# Autodesk Inventor assembly: ствол и крышка
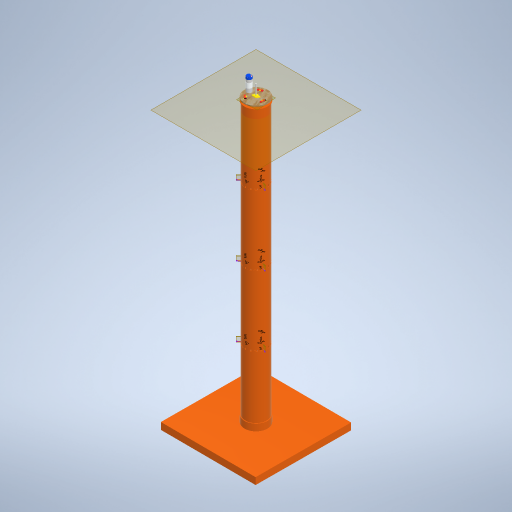
[picture p0: Inventor's stored thumbnail of the model, 512x512]
Saved by Autodesk Inventor 2023 (Build 270158000, 158)
## iProperties
Created: 2023-12-24
Part Number: ствол и крышка
Document SubType Name: Assembly
Designer: Dell
Author: Dell
## Documents named in this file (17)
- C:\Fox_Crow\Work\Crow_Sborka\ствол и крышка.iam
- C:\Fox_Crow\Work\Crow_Sborka\Поворотный механизм\Pitsco Education-739085.ipt
- C:\Fox_Crow\Work\Crow_Sborka\Поворотный механизм\Cap_pipes.ipt
- C:\Fox_Crow\Work\Crow_Sborka\Поворотный механизм\Pitsco Education-739028.ipt
- C:\Fox_Crow\Work\Crow_Sborka\Поворотный механизм\Fanerka.ipt
- C:\Fox_Crow\Work\Crow_Sborka\Поворотный механизм\Prostavka.ipt
- C:\Fox_Crow\Work\Crow_Sborka\Поворотный механизм\Det_podsh.ipt
- C:\Fox_Crow\Work\Crow_Sborka\Поворотный механизм\Podsh.ipt
- C:\Fox_Crow\Work\Crow_Sborka\Поворотный механизм\User Library-Bearing KFL08.ipt
- C:\Fox_Crow\Work\Crow_Sborka\Поворотный механизм\trubka.ipt
- C:\Users\Dell\Downloads\User Library-DC gearhead motor.ipt
- C:\Fox_Crow\Work\Crow_Sborka\Поворотный механизм\39079_TXM-Motor Shaft Hub With Set Screw.ipt
- C:\Fox_Crow\Work\Crow_Sborka\Поворотный механизм\SHF8 Горизонтальный держатель вала.ipt
- C:\Fox_Crow\Work\Crow_Sborka\Поворотный механизм\ISO 14583 — M5x16-4.8.ipt
- C:\Fox_Crow\Work\Crow_Sborka\Поворотный механизм\ISO 7046-1 - M6 x 20_ - 4.8 - H - ISO.ipt
- C:\Fox_Crow\Work\Crow_Sborka\Поворотный механизм\44260_txm torquenado dc motor.ipt
- C:\Fox_Crow\Work\Crow_Sborka\Ствол.iam
## Components (24 placed, 16 different names)
1. Pitsco Education-739085:1 — Жесткий:6, Совмещение:10, Совмещение:11, Совмещение:13, Совмещение:16
2. Cap_pipes:1 — Цилиндрический:2, Совмещение:8, Совмещение:9, Жесткий:9
3. Pitsco Education-739028:1
4. Fanerka:1 — Совмещение:9, Плоский:1, Плоский:2, Плоский:3, Цилиндрический:4, С поворотом:3, С поворотом:4, Жесткий:8
5. Prostavka:1 — Цилиндрический:2, Совмещение:8, Жесткий:5
6. User Library-Bearing KFL08:1 — С поворотом:3, С поворотом:4
7. trubka:1 — Жесткий:5, Жесткий:6, Цилиндрический:5
8. User Library-DC gearhead motor:1 — Цилиндрический:4, Жесткий:7
9. 39079_TXM-Motor Shaft Hub With Set Screw:1 — Жесткий:7
10. Винт ISO 14583:2011(E) M5x16-4.8:2
11. Винт ISO 14583:2011(E) M5x16-4.8:3
12. SHF8 Горизонтальный держатель вала:3 — Цилиндрический:5
13. ISO 7046-1 H M6 x 20 - 4.8 - H:1 — Совмещение:10
14. ISO 7046-1 H M6 x 20 - 4.8 - H:2 — Совмещение:11
15. ISO 7046-1 H M6 x 20 - 4.8 - H:3 — Совмещение:13
16. ISO 7046-1 H M6 x 20 - 4.8 - H:4 — Совмещение:16
17. 44260_txm torquenado dc motor:1 — Жесткий:8
18. Ствол:1 [sub-assembly] — Жесткий:9
19. Det_podsh:2 — С поворотом:1, Плоский:1, Плоский:2, Плоский:3
20. Podsh:1 — С поворотом:1
21. Det_podsh:3
22. Podsh:2
23. Det_podsh:4
24. Podsh:3
## Component patterns: (3 elements, first: Det_podsh:2 + Podsh:1)
## Relationships (20: Mate 6, WeldJoint 5, CylindricalJoint 3, RevoluteJoint 3, PlanarJoint 3)
- Цилиндрический:2 [CylindricalJoint]: Cap_pipes:1 ↔ Prostavka:1
- Совмещение:8 [Mate]: Cap_pipes:1 ↔ Prostavka:1
- Совмещение:9 [Mate]: Cap_pipes:1 ↔ Fanerka:1
- С поворотом:1 [RevoluteJoint]: Det_podsh:2 ↔ Podsh:1
- Плоский:1 [PlanarJoint]: Fanerka:1 ↔ Det_podsh:2
- Плоский:2 [PlanarJoint]: Fanerka:1 ↔ Det_podsh:2
- Плоский:3 [PlanarJoint]: Fanerka:1 ↔ Det_podsh:2
- Жесткий:5 [WeldJoint]: Prostavka:1 ↔ trubka:1
- Жесткий:6 [WeldJoint]: Pitsco Education-739085:1 ↔ trubka:1
- Цилиндрический:4 [CylindricalJoint]: Fanerka:1 ↔ User Library-DC gearhead motor:1
- Жесткий:7 [WeldJoint]: User Library-DC gearhead motor:1 ↔ 39079_TXM-Motor Shaft Hub With Set Screw:1
- С поворотом:3 [RevoluteJoint]: Fanerka:1 ↔ User Library-Bearing KFL08:1
- С поворотом:4 [RevoluteJoint]: Fanerka:1 ↔ User Library-Bearing KFL08:1
- Цилиндрический:5 [CylindricalJoint]: trubka:1 ↔ SHF8 Горизонтальный держатель вала:3
- Совмещение:10 [Mate]: Pitsco Education-739085:1 ↔ ISO 7046-1 H M6 x 20 - 4.8 - H:1
- Совмещение:11 [Mate]: Pitsco Education-739085:1 ↔ ISO 7046-1 H M6 x 20 - 4.8 - H:2
- Совмещение:13 [Mate]: Pitsco Education-739085:1 ↔ ISO 7046-1 H M6 x 20 - 4.8 - H:3
- Совмещение:16 [Mate]: Pitsco Education-739085:1 ↔ ISO 7046-1 H M6 x 20 - 4.8 - H:4
- Жесткий:8 [WeldJoint]: Fanerka:1 ↔ 44260_txm torquenado dc motor:1
- Жесткий:9 [WeldJoint]: Cap_pipes:1 ↔ Ствол:1
